# Autodesk Inventor assembly: Laser_Mount
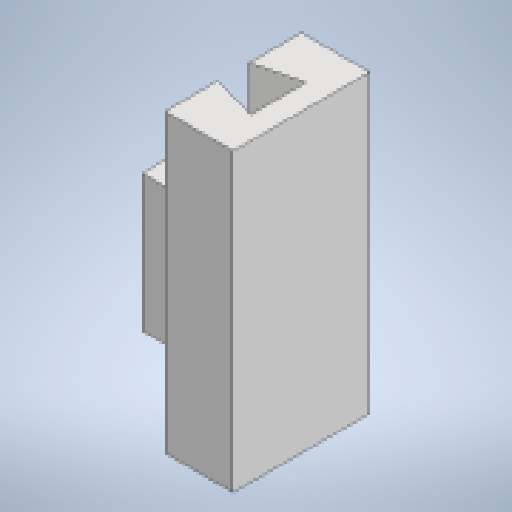
[picture p0: Inventor's stored thumbnail of the model, 512x512]
Saved by Autodesk Inventor 2023 (Build 270158000, 158)
## iProperties
Created: 2024-01-06
Part Number: Laser_Mount
Document SubType Name: Assembly
Designer: a laptop
Author: a laptop
## Documents named in this file (3)
- C:\Users\a laptop\Desktop\CNC_Project\Laser_Mount.iam
- C:\Users\a laptop\Desktop\CNC_Project\Laser_Base.ipt
- C:\Users\a laptop\Desktop\CNC_Project\Laser_Mount.ipt
## Components (2 placed, 2 different names)
1. Laser_Base:1 — Mate:1, Flush:1
2. Laser_Mount:1 — Mate:1, Flush:1
## Relationships (2: Mate 1, Flush 1)
- Mate:1: Laser_Base:1 ↔ Laser_Mount:1
- Flush:1: Laser_Base:1 ↔ Laser_Mount:1
